# Autodesk Inventor assembly: wheel_ass_1
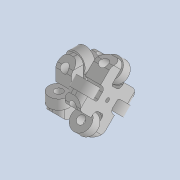
[picture p0: Inventor's stored thumbnail of the model, 180x180]
Saved by Autodesk Inventor 2020 (Build 240168000, 168)
## iProperties
Created: 2021-12-22
Part Number: wheel_ass_1
Document SubType Name: Assembly
Designer: Shuang Peng
Author: Shuang Peng
## Documents named in this file (2)
- D:\projects-3\soft module robot\hardware\diff module 3\wheel_ass_1.iam
- D:\projects-3\soft module robot\hardware\diff module 3\wheel_ass_s1.iam
## Components (2 placed, 1 different names)
1. wheel_ass_s1:1 [sub-assembly] — Angle:1, Insert:1
2. wheel_ass_s1:2 [sub-assembly] — Angle:1, Insert:1
## Relationships (2: Angle 1, Insert 1)
- Angle:1 (45 deg): wheel_ass_s1:1 ↔ wheel_ass_s1:2
- Insert:1 (1 mm): wheel_ass_s1:1 ↔ wheel_ass_s1:2
